# Autodesk Inventor assembly: ASY SLM 1690 Filter legs D1000
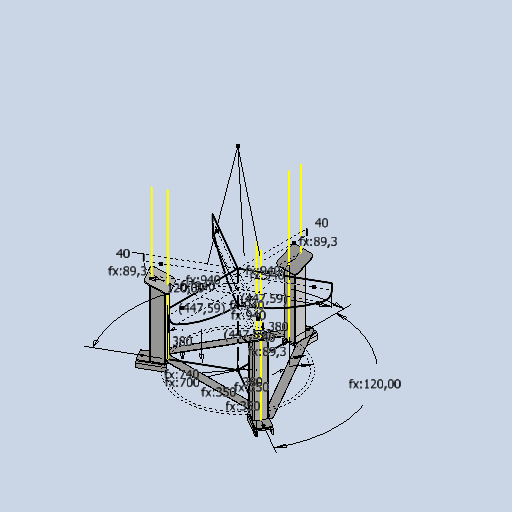
[picture p0: Inventor's stored thumbnail of the model, 512x512]
Saved by Autodesk Inventor 2025 (Build 290162010, 162A)
## iProperties
Created: 2025-02-20
Part Number: ASY SLM 1690 Filter legs D1000
Document SubType Name: Assembly
Designer: user
Mass: 20950.1 g
Surface Area: 14148.6 cm^2
Volume: 2651.55 cm^3
Density: 7.9011 g/cm^3
Author: user
## Documents named in this file (7)
- C:\Users\admin\Yandex.Disk\home pc\Inventor\SLM-Salemal\ASY PNS 1690 Filter legs D1000.iam
- C:\Users\admin\Yandex.Disk\home pc\Inventor\SLM-Salemal\PNS 1692 Leg tube.ipt
- C:\Users\admin\Yandex.Disk\home pc\Inventor\SLM-Salemal\PNS 1693 leg sketch.ipt
- C:\Users\admin\Yandex.Disk\home pc\Inventor\SLM-Salemal\PNS 1694 leg plate for filter.ipt
- C:\Users\admin\Yandex.Disk\home pc\Inventor\SLM-Salemal\PNS 1695 leg floor plate.ipt
- C:\Users\admin\Yandex.Disk\home pc\Inventor\SLM-Salemal\PNS 1785 leg floor channel.ipt
- C:\Users\admin\Yandex.Disk\home pc\Inventor\SLM-Salemal\PNS 1696 leg floor pattern.ipt
## Components (14 placed, 6 different names)
1. PNS 1692 Leg tube.ipt:1 — Mate:2, Mate:8, Tangent:2, Rigid:2, Rigid:5
2. PNS 1692 Leg tube.ipt:2 — Mate:4, Mate:7, Tangent:3, Rigid:1, Rigid:4
3. PNS 1692 Leg tube.ipt:3 — Mate:3, Mate:6, Tangent:1, Rigid:3, Rigid:6
4. PNS 1693 leg sketch.ipt:1 — Mate:6, Tangent:1, Mate:7, Mate:8, Tangent:2, Tangent:3
5. PNS 1694 leg plate for filter.ipt:1 — Rigid:1
6. PNS 1694 leg plate for filter.ipt:2 — Rigid:2
7. PNS 1694 leg plate for filter.ipt:3 — Rigid:3
8. PNS 1695 leg floor plate.ipt:1 — Rigid:4, Rigid:10, Rotational:4
9. PNS 1695 leg floor plate.ipt:2 — Rigid:5, Rigid:7
10. PNS 1695 leg floor plate.ipt:3 — Rigid:6, Rigid:9
11. PNS 1785 leg floor channel.ipt:1 — Rigid:10
12. PNS 1785 leg floor channel.ipt:2 — Rigid:9
13. PNS 1785 leg floor channel.ipt:3 — Rigid:7
14. PNS 1696 leg floor pattern.ipt:1 — Rotational:4
## Relationships (19: WeldJoint 9, Mate 6, Tangent 3, RevoluteJoint 1)
- Mate:2: PNS 1692 Leg tube.ipt:1
- Mate:3: PNS 1692 Leg tube.ipt:3
- Mate:4: PNS 1692 Leg tube.ipt:2
- Mate:6: PNS 1692 Leg tube.ipt:3 ↔ PNS 1693 leg sketch.ipt:1
- Tangent:1: PNS 1692 Leg tube.ipt:3 ↔ PNS 1693 leg sketch.ipt:1
- Mate:7: PNS 1692 Leg tube.ipt:2 ↔ PNS 1693 leg sketch.ipt:1
- Mate:8: PNS 1692 Leg tube.ipt:1 ↔ PNS 1693 leg sketch.ipt:1
- Tangent:2: PNS 1692 Leg tube.ipt:1 ↔ PNS 1693 leg sketch.ipt:1
- Tangent:3: PNS 1692 Leg tube.ipt:2 ↔ PNS 1693 leg sketch.ipt:1
- Rigid:1 [WeldJoint]: PNS 1692 Leg tube.ipt:2 ↔ PNS 1694 leg plate for filter.ipt:1
- Rigid:2 [WeldJoint]: PNS 1692 Leg tube.ipt:1 ↔ PNS 1694 leg plate for filter.ipt:2
- Rigid:3 [WeldJoint]: PNS 1692 Leg tube.ipt:3 ↔ PNS 1694 leg plate for filter.ipt:3
- Rigid:4 [WeldJoint]: PNS 1692 Leg tube.ipt:2 ↔ PNS 1695 leg floor plate.ipt:1
- Rigid:5 [WeldJoint]: PNS 1692 Leg tube.ipt:1 ↔ PNS 1695 leg floor plate.ipt:2
- Rigid:6 [WeldJoint]: PNS 1692 Leg tube.ipt:3 ↔ PNS 1695 leg floor plate.ipt:3
- Rigid:7 [WeldJoint]: PNS 1695 leg floor plate.ipt:2 ↔ PNS 1785 leg floor channel.ipt:3
- Rigid:9 [WeldJoint]: PNS 1695 leg floor plate.ipt:3 ↔ PNS 1785 leg floor channel.ipt:2
- Rigid:10 [WeldJoint]: PNS 1695 leg floor plate.ipt:1 ↔ PNS 1785 leg floor channel.ipt:1
- Rotational:4 [RevoluteJoint]: PNS 1695 leg floor plate.ipt:1 ↔ PNS 1696 leg floor pattern.ipt:1
